# Autodesk Inventor assembly: 5211900 DSNU-S-12-30-P-A-MQ---(0)
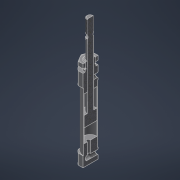
[picture p0: Inventor's stored thumbnail of the model, 180x180]
Saved by Autodesk Inventor 2022 (Build 260153000, 153)
## iProperties
Created: 2023-03-28
Part Number: 5211900 DSNU-S-12-30-P-A-MQ---(0)
Catalog Web Link: www.cadenas.de
Description: DSNU-S-round cylinder
Vendor: FESTO
Document SubType Name: Assembly
Designer: psAdmin
Manufacturer: FESTO
Mass: 87 g
Surface Area: 88.6067 cm^2
Volume: 10.2389 cm^3
Density: 8.49697 g/cm^3
Category: PARTsolutions
Company: FESTO
PSOL_IDENT_0: {ATYP=ASSISTANT},{DATA=script=$CADENAS_DATA/23d-libs/festo/webfesto.vbb&M_FAMILY=DSNU&M_GROUP=01&M_P
PSOL_IDENT_1: ARTNO=5211900&IDCODE1=DSNU-S-12-30-P-A-MQ&IDCODE2=&customer_number_cns=&MATES=1&LOD=HI&LOCKERP=0&SIN
PSOL_IDENT_2: GLEPART=1}
NB: 5211900 DSNU-S-12-30-P-A-MQ---(0)
NN: DSNU-S
NT: round cylinder
NBSYN: $TNR. $TYP.---($HUBST.)
LINA: 5211900 DSNU-S-12-30-P-A-MQ
CATALOG: Festo
TNR: 5211900
TYP: DSNU-S-12-30-P-A-MQ
KDM: 12
HUB: 30
HUBST: 0
DA: P
PE: A
ZYL: MQ
AM: 16
B: 10
BE: M10x1
BF: 8.1
D: 16
D1: 14
D4: 13.3
EE: M5
G: 9.65
G1: 11.95
KK: M6
KV: 14
KW: 4
L2: 75.85
MM: 6
PL: 6
PL1: 8
SW: 5
VD: 1.5
WF: 13
ZJ: 89.3
CNSMASSEXACT: 0.087
SUPPLIER: FESTO
ARTICLENO: 5211900 DSNU-S-12-30-P-A-MQ---(0)
BOMINFO: 5211900 DSNU-S-12-30-P-A-MQ
CREATOR: CADENAS GmbH
Title: 5211900 DSNU-S-12-30-P-A-MQ
Author: Cadenas PARTsolutions
Comments: round cylinder
## Documents named in this file (4)
- D:\Pulpit\dni otwarte\5211900 DSNU-S-12-30-P-A-MQ---(0).iam
- D:\Pulpit\dni otwarte\8112003 DSNU-S-12-30-P-MQ---(C).ipt
- D:\Pulpit\dni otwarte\8112003 DSNU-S-12-30-P---(P).ipt
- D:\Pulpit\dni otwarte\5362901 M10x1.ipt
## Components (3 placed, 3 different names)
1. 8112003 DSNU-S-12-30-P-MQ---(C):1 — to_piston_XY@1 <-> ANBAU_XY@2, to_piston_Z@1 <-> ANBAU_Z@2, to_piston_YZ@1 <-> ANBAU_YZ@2, to_nut_XY@1 <-> ANBAU_XY@3, to_nut_Z@1 <-> ANBAU_Z@3, to_nut_YZ@1 <-> ANBAU_YZ@3
2. 8112003 DSNU-S-12-30-P---(P):1 — to_piston_XY@1 <-> ANBAU_XY@2, to_piston_Z@1 <-> ANBAU_Z@2, to_piston_YZ@1 <-> ANBAU_YZ@2
3. 5362901 M10x1:1 — to_nut_XY@1 <-> ANBAU_XY@3, to_nut_Z@1 <-> ANBAU_Z@3, to_nut_YZ@1 <-> ANBAU_YZ@3
## Relationships (6: Mate 4, Angle 2)
- to_piston_XY@1 <-> ANBAU_XY@2 [Mate]: 8112003 DSNU-S-12-30-P-MQ---(C):1 ↔ 8112003 DSNU-S-12-30-P---(P):1
- to_piston_Z@1 <-> ANBAU_Z@2 [Mate]: 8112003 DSNU-S-12-30-P-MQ---(C):1 ↔ 8112003 DSNU-S-12-30-P---(P):1
- to_piston_YZ@1 <-> ANBAU_YZ@2 [Angle] (0 deg): 8112003 DSNU-S-12-30-P-MQ---(C):1 ↔ 8112003 DSNU-S-12-30-P---(P):1
- to_nut_XY@1 <-> ANBAU_XY@3 [Mate]: 8112003 DSNU-S-12-30-P-MQ---(C):1 ↔ 5362901 M10x1:1
- to_nut_Z@1 <-> ANBAU_Z@3 [Mate]: 8112003 DSNU-S-12-30-P-MQ---(C):1 ↔ 5362901 M10x1:1
- to_nut_YZ@1 <-> ANBAU_YZ@3 [Angle] (0 deg): 8112003 DSNU-S-12-30-P-MQ---(C):1 ↔ 5362901 M10x1:1
